# Autodesk Inventor assembly: 000-belt_liner_v1
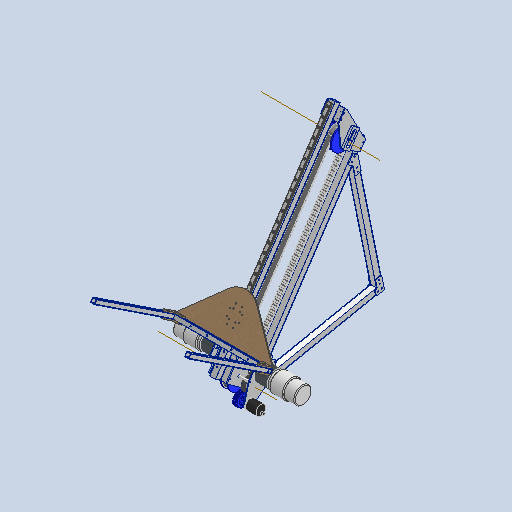
[picture p0: Inventor's stored thumbnail of the model, 512x512]
Saved by Autodesk Inventor 2025.1 (Build 291241000, 241)
## iProperties
Created: 2024-12-08
Part Number: 000-belt_liner_v1
Document SubType Name: Assembly
Designer: haruy
Author: haruy
## Documents named in this file (35)
- C:\Users\haruy\Documents\ロボコン\NHK2025\cad\nagahisa\belt_liner\000-belt_liner_v1.iam
- C:\Users\haruy\Documents\ロボコン\NHK2025\cad\nagahisa\belt_liner\belt_liner_v1_ASP_Base.ipt
- C:\Users\haruy\Documents\ロボコン\NHK2025\cad\nagahisa\belt_liner\SSE2B-MX10-455.iam
- C:\Users\haruy\Documents\ロボコン\NHK2025\cad\nagahisa\belt_liner\belt_liner_v1_Plate_1.ipt
- C:\Users\haruy\Documents\ロボコン\NHK2025\cad\nagahisa\belt_liner\belt_liner_v1_Plate_2.ipt
- C:\Users\haruy\Documents\ロボコン\NHK2025\cad\nagahisa\belt_liner\belt_liner_v1_Plate_3.ipt
- C:\Users\haruy\Documents\ロボコン\NHK2025\cad\000_parts\ベアリング\10\bear_10_15_sn.ipt
- C:\Users\haruy\Documents\ロボコン\NHK2025\cad\nagahisa\belt_liner\belt_liner_v1_shaft_spesa-25.ipt
- C:\Users\haruy\Documents\ロボコン\NHK2025\cad\nagahisa\belt_liner\belt_liner_v1_Plate_4.ipt
- C:\Users\haruy\Documents\ロボコン\NHK2025\cad\nagahisa\belt_liner\belt_liner_v1_Plate_5.ipt
- C:\Users\haruy\Documents\ロボコン\NHK2025\cad\000_parts\モーター\RS-775GM_004GH.iam
- C:\Users\haruy\Documents\ロボコン\NHK2025\cad\000_parts\エンコーダー\encoder v2.ipt
- C:\Users\haruy\Documents\ロボコン\NHK2025\cad\nagahisa\belt_liner\belt_liner_v1_Plate_6.ipt
- C:\Users\haruy\Documents\ロボコン\NHK2025\cad\nagahisa\belt_liner\belt_liner_v1_Plate_7.ipt
- C:\Users\haruy\Documents\ロボコン\NHK2025\cad\nagahisa\belt_liner\belt_liner_v1_Plate_8.ipt
- C:\Users\haruy\Documents\ロボコン\NHK2025\cad\nagahisa\belt_liner\belt_liner_v1_Plate_9.ipt
- C:\Users\haruy\Documents\ロボコン\NHK2025\cad\nagahisa\belt_liner\000-belt_liner_v1\デザイン アクセラレータ\歯付きベルト伝達1.iam
- C:\Users\haruy\Documents\ロボコン\NHK2025\cad\nagahisa\belt_liner\belt_liner_v1_shaft-54.ipt
- C:\Users\haruy\Documents\ロボコン\NHK2025\cad\nagahisa\belt_liner\SCSWJ10-6.iam
- C:\Users\haruy\Documents\ロボコン\NHK2025\cad\nagahisa\belt_liner\belt_liner_v1_shaft-84.ipt
- C:\Users\haruy\Documents\ロボコン\NHK2025\cad\nagahisa\belt_liner\000-belt_liner_v1\デザイン アクセラレータ\平歯車1.iam
- C:\Users\haruy\Documents\ロボコン\NHK2025\cad\nagahisa\belt_liner\000-belt_liner_v1\デザイン アクセラレータ\平歯車1_MIR.iam
- C:\Users\haruy\Documents\ロボコン\NHK2025\cad\nagahisa\belt_liner\belt_liner_v1_3DP_spesa-1.ipt
- C:\Users\haruy\Documents\ロボコン\NHK2025\cad\nagahisa\belt_liner\belt_liner_v1_3DP_spesa-2.ipt
- C:\Users\haruy\Documents\ロボコン\NHK2025\cad\nagahisa\belt_liner\belt_liner_v1_MDF_throw_plate.ipt
- C:\Users\haruy\Documents\ロボコン\NHK2025\cad\nagahisa\belt_liner\belt_liner_v1_Plate_10.ipt
- C:\Users\haruy\Documents\ロボコン\NHK2025\cad\nagahisa\belt_liner\belt_liner_v1_Plate_11.ipt
- C:\Users\haruy\Documents\ロボコン\NHK2025\cad\nagahisa\belt_liner\belt_liner_v1_Plate_12.ipt
- C:\Users\haruy\Documents\ロボコン\NHK2025\cad\nagahisa\belt_liner\belt_liner_v1_Plate_13.ipt
- C:\Users\haruy\Documents\ロボコン\NHK2025\cad\nagahisa\belt_liner\belt_liner_v1_ASP_Ca.ipt
- C:\Users\haruy\Documents\ロボコン\NHK2025\cad\nagahisa\belt_liner\belt_liner_v1_MDF_F_1.ipt
- C:\Users\haruy\Documents\ロボコン\NHK2025\cad\nagahisa\belt_liner\belt_liner_v1_Plate_14.ipt
- C:\Users\haruy\Documents\ロボコン\NHK2025\cad\nagahisa\belt_liner\belt_liner_v1_Plate_15.ipt
- C:\Users\haruy\Documents\ロボコン\NHK2025\cad\nagahisa\belt_liner\000-belt_liner_v1\デザイン アクセラレータ\平歯車2.iam
- C:\Users\haruy\Documents\ロボコン\NHK2025\cad\nagahisa\dribl\R2-Rzvector\RZvector-v1-3DP-E-F.ipt
## Components (59 placed, 33 different names)
1. belt_liner_v1_ASP_Base:1 — 挿入:1, 挿入:2, 挿入:3, 挿入:4, 挿入:5, 挿入:6, 挿入:28, 挿入:29, 挿入:30, 挿入:31, フラッシュ:1, 挿入:62, 挿入:63, 挿入:64, 挿入:65, 挿入:66, 挿入:67, 挿入:68, 挿入:69, 挿入:70, 挿入:71, 挿入:72, 挿入:73
2. SSE2B-MX10-455:1 [sub-assembly] — 挿入:1, 挿入:2, 挿入:51, 挿入:52
3. belt_liner_v1_Plate_1:1 — 挿入:3, 挿入:4
4. belt_liner_v1_Plate_2:1 — 挿入:5, 挿入:6, 挿入:7, 挿入:8, 挿入:9, 挿入:10
5. belt_liner_v1_Plate_3:1 — 挿入:7, 挿入:8, 挿入:12, 挿入:89, 挿入:90, 挿入:91, 挿入:92
6. belt_liner_v1_Plate_3:2 — 挿入:9, 挿入:10, 挿入:11, 挿入:95, 挿入:96, 挿入:97, 挿入:98
7. bear_10_15_sn:1 — 挿入:11, 挿入:55
8. bear_10_15_sn:2 — 挿入:12, 挿入:50
9. belt_liner_v1_Plate_4:1 — 挿入:25, 挿入:27, 挿入:86, 挿入:93, 挿入:94
10. belt_liner_v1_Plate_5:1 — 挿入:26, 挿入:99, 挿入:100
11. RS-775GM_004GH:1 [sub-assembly] — 挿入:25
12. RS-775GM_004GH:2 [sub-assembly] — 挿入:26, メイト:3
13. encoder v2:1 — 挿入:27
14. belt_liner_v1_Plate_6:1 — 挿入:28, 挿入:29, 挿入:32, 挿入:34, 挿入:35
15. belt_liner_v1_Plate_7:1 — 挿入:30, 挿入:31, 挿入:33
16. belt_liner_v1_Plate_8:1 — 挿入:32, 挿入:33, 挿入:36, 挿入:37
17. belt_liner_v1_Plate_8:2 — 挿入:34, 挿入:35, 挿入:38, 挿入:39
18. belt_liner_v1_Plate_9:1 — 挿入:38, 挿入:39
19. belt_liner_v1_Plate_9:2 — 挿入:36, 挿入:37, 正接:1
20. 歯付きベルト伝達:1 [sub-assembly] — 挿入:40, 挿入:41, 挿入:43, 挿入:49, メイト:5, メイト:6
21. bear_10_15_sn:3 — 挿入:40, 挿入:42, 挿入:47
22. bear_10_15_sn:4 — 挿入:41, 挿入:48
23. belt_liner_v1_shaft-54:1 — 挿入:42, 正接:1
24. SCSWJ10-6:1 [sub-assembly] — 挿入:43, 挿入:44
25. belt_liner_v1_shaft-84:1 — 挿入:44, 挿入:45, 挿入:46, メイト:1
26. SCSWJ10-6:2 [sub-assembly] — 挿入:45
27. SCSWJ10-6:3 [sub-assembly] — 挿入:46, メイト:2
28. 平歯車:1 [sub-assembly] — メイト:1, メイト:2, メイト:3
29. 平歯車1_MIR:1 [sub-assembly]
30. belt_liner_v1_3DP_spesa-1:1 — 挿入:47
31. belt_liner_v1_3DP_spesa-1:2 — 挿入:48
32. belt_liner_v1_3DP_spesa-1:3 — 挿入:49, 挿入:55
33. belt_liner_v1_3DP_spesa-2:1 — 挿入:50
34. belt_liner_v1_MDF_throw_plate:1 — 挿入:51, 挿入:52, 挿入:58, 挿入:59, 挿入:60, 挿入:61, 挿入:74, 挿入:75
35. belt_liner_v1_Plate_10:1 — 挿入:58, 挿入:61
36. belt_liner_v1_Plate_10:2 — 挿入:59, 挿入:60
37. belt_liner_v1_Plate_11:1 — 挿入:64, 挿入:65
38. belt_liner_v1_Plate_11:2 — 挿入:62, 挿入:63
39. belt_liner_v1_Plate_12:1 — 挿入:68, 挿入:69
40. belt_liner_v1_Plate_12:2 — 挿入:66, 挿入:67
41. belt_liner_v1_Plate_13:1 — 挿入:72, 挿入:73
42. belt_liner_v1_Plate_13:2 — 挿入:70, 挿入:71
43. belt_liner_v1_ASP_Ca:1 — 挿入:74, 挿入:75, 挿入:76, 挿入:77, 挿入:78, 挿入:79, 挿入:80, 挿入:81, 挿入:82, 挿入:83
44. belt_liner_v1_MDF_F_1:1 — 挿入:80, 挿入:81
45. belt_liner_v1_MDF_F_1:2 — 挿入:76, 挿入:77
46. belt_liner_v1_MDF_F_1:3 — 挿入:78, 挿入:79
47. belt_liner_v1_MDF_F_1:4 — 挿入:82, 挿入:83
48. belt_liner_v1_Plate_14:1 — 挿入:84, 挿入:85
49. belt_liner_v1_Plate_15:1 — 挿入:84, 挿入:85, メイト:5, メイト:6
50. 平歯車:2 [sub-assembly] — 挿入:86, 挿入:87, 挿入:88
51. RZvector-v1-3DP-E-F:1 — 挿入:87, 挿入:88
52. belt_liner_v1_shaft_spesa-25:1 — 挿入:90
53. belt_liner_v1_shaft_spesa-25:2 — 挿入:91, 挿入:93
54. belt_liner_v1_shaft_spesa-25:3 — 挿入:92
55. belt_liner_v1_shaft_spesa-25:4 — 挿入:89, 挿入:94
56. belt_liner_v1_shaft_spesa-25:5 — 挿入:96, 挿入:99
57. belt_liner_v1_shaft_spesa-25:6 — 挿入:98
58. belt_liner_v1_shaft_spesa-25:7 — 挿入:97
59. belt_liner_v1_shaft_spesa-25:8 — 挿入:95, 挿入:100
## Relationships (91: Insert 84, Mate 5, Flush 1, Tangent 1)
- 挿入:1 [Insert]: belt_liner_v1_ASP_Base:1 ↔ SSE2B-MX10-455:1
- 挿入:2 [Insert]: belt_liner_v1_ASP_Base:1 ↔ SSE2B-MX10-455:1
- 挿入:3 [Insert]: belt_liner_v1_ASP_Base:1 ↔ belt_liner_v1_Plate_1:1
- 挿入:4 [Insert]: belt_liner_v1_ASP_Base:1 ↔ belt_liner_v1_Plate_1:1
- 挿入:5 [Insert]: belt_liner_v1_ASP_Base:1 ↔ belt_liner_v1_Plate_2:1
- 挿入:6 [Insert]: belt_liner_v1_ASP_Base:1 ↔ belt_liner_v1_Plate_2:1
- 挿入:7 [Insert]: belt_liner_v1_Plate_2:1 ↔ belt_liner_v1_Plate_3:1
- 挿入:8 [Insert]: belt_liner_v1_Plate_2:1 ↔ belt_liner_v1_Plate_3:1
- 挿入:9 [Insert]: belt_liner_v1_Plate_2:1 ↔ belt_liner_v1_Plate_3:2
- 挿入:10 [Insert]: belt_liner_v1_Plate_2:1 ↔ belt_liner_v1_Plate_3:2
- 挿入:11 [Insert]: belt_liner_v1_Plate_3:2 ↔ bear_10_15_sn:1
- 挿入:12 [Insert]: belt_liner_v1_Plate_3:1 ↔ bear_10_15_sn:2
- 挿入:25 [Insert]: belt_liner_v1_Plate_4:1 ↔ RS-775GM_004GH:1
- 挿入:26 [Insert]: belt_liner_v1_Plate_5:1 ↔ RS-775GM_004GH:2
- 挿入:27 [Insert]: belt_liner_v1_Plate_4:1 ↔ encoder v2:1
- 挿入:28 [Insert]: belt_liner_v1_ASP_Base:1 ↔ belt_liner_v1_Plate_6:1
- 挿入:29 [Insert]: belt_liner_v1_ASP_Base:1 ↔ belt_liner_v1_Plate_6:1
- 挿入:30 [Insert]: belt_liner_v1_ASP_Base:1 ↔ belt_liner_v1_Plate_7:1
- 挿入:31 [Insert]: belt_liner_v1_ASP_Base:1 ↔ belt_liner_v1_Plate_7:1
- 挿入:32 [Insert]: belt_liner_v1_Plate_6:1 ↔ belt_liner_v1_Plate_8:1
- 挿入:33 [Insert]: belt_liner_v1_Plate_7:1 ↔ belt_liner_v1_Plate_8:1
- 挿入:34 [Insert]: belt_liner_v1_Plate_6:1 ↔ belt_liner_v1_Plate_8:2
- 挿入:35 [Insert]: belt_liner_v1_Plate_6:1 ↔ belt_liner_v1_Plate_8:2
- 挿入:36 [Insert]: belt_liner_v1_Plate_8:1 ↔ belt_liner_v1_Plate_9:2
- 挿入:37 [Insert]: belt_liner_v1_Plate_8:1 ↔ belt_liner_v1_Plate_9:2
- 挿入:38 [Insert]: belt_liner_v1_Plate_8:2 ↔ belt_liner_v1_Plate_9:1
- 挿入:39 [Insert]: belt_liner_v1_Plate_8:2 ↔ belt_liner_v1_Plate_9:1
- フラッシュ:1 [Flush] (-7.5 mm): belt_liner_v1_ASP_Base:1
- 挿入:40 [Insert]: 歯付きベルト伝達:1 ↔ bear_10_15_sn:3
- 挿入:41 [Insert]: 歯付きベルト伝達:1 ↔ bear_10_15_sn:4
- 挿入:42 [Insert] (-16.5 mm): bear_10_15_sn:3 ↔ belt_liner_v1_shaft-54:1
- 挿入:43 [Insert]: 歯付きベルト伝達:1 ↔ SCSWJ10-6:1
- 挿入:44 [Insert] (-26.5 mm): SCSWJ10-6:1 ↔ belt_liner_v1_shaft-84:1
- 挿入:45 [Insert]: belt_liner_v1_shaft-84:1 ↔ SCSWJ10-6:2
- 挿入:46 [Insert]: belt_liner_v1_shaft-84:1 ↔ SCSWJ10-6:3
- メイト:1 [Mate]: belt_liner_v1_shaft-84:1 ↔ 平歯車:1
- メイト:2 [Mate]: SCSWJ10-6:3 ↔ 平歯車:1
- メイト:3 [Mate]: RS-775GM_004GH:2 ↔ 平歯車:1
- 挿入:47 [Insert]: bear_10_15_sn:3 ↔ belt_liner_v1_3DP_spesa-1:1
- 挿入:48 [Insert]: bear_10_15_sn:4 ↔ belt_liner_v1_3DP_spesa-1:2
- 挿入:49 [Insert]: 歯付きベルト伝達:1 ↔ belt_liner_v1_3DP_spesa-1:3
- 挿入:50 [Insert]: bear_10_15_sn:2 ↔ belt_liner_v1_3DP_spesa-2:1
- 挿入:51 [Insert]: SSE2B-MX10-455:1 ↔ belt_liner_v1_MDF_throw_plate:1
- 挿入:52 [Insert]: SSE2B-MX10-455:1 ↔ belt_liner_v1_MDF_throw_plate:1
- 挿入:55 [Insert]: bear_10_15_sn:1 ↔ belt_liner_v1_3DP_spesa-1:3
- 正接:1 [Tangent]: belt_liner_v1_Plate_9:2 ↔ belt_liner_v1_shaft-54:1
- 挿入:58 [Insert]: belt_liner_v1_MDF_throw_plate:1 ↔ belt_liner_v1_Plate_10:1
- 挿入:59 [Insert]: belt_liner_v1_MDF_throw_plate:1 ↔ belt_liner_v1_Plate_10:2
- 挿入:60 [Insert]: belt_liner_v1_MDF_throw_plate:1 ↔ belt_liner_v1_Plate_10:2
- 挿入:61 [Insert]: belt_liner_v1_MDF_throw_plate:1 ↔ belt_liner_v1_Plate_10:1
- 挿入:62 [Insert]: belt_liner_v1_ASP_Base:1 ↔ belt_liner_v1_Plate_11:2
- 挿入:63 [Insert]: belt_liner_v1_ASP_Base:1 ↔ belt_liner_v1_Plate_11:2
- 挿入:64 [Insert]: belt_liner_v1_ASP_Base:1 ↔ belt_liner_v1_Plate_11:1
- 挿入:65 [Insert]: belt_liner_v1_ASP_Base:1 ↔ belt_liner_v1_Plate_11:1
- 挿入:66 [Insert]: belt_liner_v1_ASP_Base:1 ↔ belt_liner_v1_Plate_12:2
- 挿入:67 [Insert]: belt_liner_v1_ASP_Base:1 ↔ belt_liner_v1_Plate_12:2
- 挿入:68 [Insert]: belt_liner_v1_ASP_Base:1 ↔ belt_liner_v1_Plate_12:1
- 挿入:69 [Insert]: belt_liner_v1_ASP_Base:1 ↔ belt_liner_v1_Plate_12:1
- 挿入:70 [Insert]: belt_liner_v1_ASP_Base:1 ↔ belt_liner_v1_Plate_13:2
- 挿入:71 [Insert]: belt_liner_v1_ASP_Base:1 ↔ belt_liner_v1_Plate_13:2
- 挿入:72 [Insert]: belt_liner_v1_ASP_Base:1 ↔ belt_liner_v1_Plate_13:1
- 挿入:73 [Insert]: belt_liner_v1_ASP_Base:1 ↔ belt_liner_v1_Plate_13:1
- 挿入:74 [Insert]: belt_liner_v1_MDF_throw_plate:1 ↔ belt_liner_v1_ASP_Ca:1
- 挿入:75 [Insert]: belt_liner_v1_MDF_throw_plate:1 ↔ belt_liner_v1_ASP_Ca:1
- 挿入:76 [Insert]: belt_liner_v1_ASP_Ca:1 ↔ belt_liner_v1_MDF_F_1:2
- 挿入:77 [Insert]: belt_liner_v1_ASP_Ca:1 ↔ belt_liner_v1_MDF_F_1:2
- 挿入:78 [Insert]: belt_liner_v1_ASP_Ca:1 ↔ belt_liner_v1_MDF_F_1:3
- 挿入:79 [Insert]: belt_liner_v1_ASP_Ca:1 ↔ belt_liner_v1_MDF_F_1:3
- 挿入:80 [Insert]: belt_liner_v1_ASP_Ca:1 ↔ belt_liner_v1_MDF_F_1:1
- 挿入:81 [Insert]: belt_liner_v1_ASP_Ca:1 ↔ belt_liner_v1_MDF_F_1:1
- 挿入:82 [Insert]: belt_liner_v1_ASP_Ca:1 ↔ belt_liner_v1_MDF_F_1:4
- 挿入:83 [Insert]: belt_liner_v1_ASP_Ca:1 ↔ belt_liner_v1_MDF_F_1:4
- 挿入:84 [Insert]: belt_liner_v1_Plate_14:1 ↔ belt_liner_v1_Plate_15:1
- 挿入:85 [Insert]: belt_liner_v1_Plate_14:1 ↔ belt_liner_v1_Plate_15:1
- メイト:5 [Mate]: 歯付きベルト伝達:1 ↔ belt_liner_v1_Plate_15:1
- メイト:6 [Mate]: 歯付きベルト伝達:1 ↔ belt_liner_v1_Plate_15:1
- 挿入:86 [Insert] (3 mm): belt_liner_v1_Plate_4:1 ↔ 平歯車:2
- 挿入:87 [Insert]: 平歯車:2 ↔ RZvector-v1-3DP-E-F:1
- 挿入:88 [Insert]: 平歯車:2 ↔ RZvector-v1-3DP-E-F:1
- 挿入:89 [Insert]: belt_liner_v1_Plate_3:1 ↔ belt_liner_v1_shaft_spesa-25:4
- 挿入:90 [Insert]: belt_liner_v1_Plate_3:1 ↔ belt_liner_v1_shaft_spesa-25:1
- 挿入:91 [Insert]: belt_liner_v1_Plate_3:1 ↔ belt_liner_v1_shaft_spesa-25:2
- 挿入:92 [Insert]: belt_liner_v1_Plate_3:1 ↔ belt_liner_v1_shaft_spesa-25:3
- 挿入:93 [Insert]: belt_liner_v1_Plate_4:1 ↔ belt_liner_v1_shaft_spesa-25:2
- 挿入:94 [Insert]: belt_liner_v1_Plate_4:1 ↔ belt_liner_v1_shaft_spesa-25:4
- 挿入:95 [Insert]: belt_liner_v1_Plate_3:2 ↔ belt_liner_v1_shaft_spesa-25:8
- 挿入:96 [Insert]: belt_liner_v1_Plate_3:2 ↔ belt_liner_v1_shaft_spesa-25:5
- 挿入:97 [Insert]: belt_liner_v1_Plate_3:2 ↔ belt_liner_v1_shaft_spesa-25:7
- 挿入:98 [Insert]: belt_liner_v1_Plate_3:2 ↔ belt_liner_v1_shaft_spesa-25:6
- 挿入:99 [Insert]: belt_liner_v1_Plate_5:1 ↔ belt_liner_v1_shaft_spesa-25:5
- 挿入:100 [Insert]: belt_liner_v1_Plate_5:1 ↔ belt_liner_v1_shaft_spesa-25:8
